# Autodesk Inventor assembly: 217-2792-001 Rev1
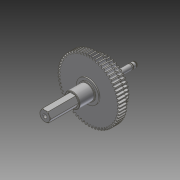
[picture p0: Inventor's stored thumbnail of the model, 180x180]
Saved by Autodesk Inventor 2014 SP1 (Build 180222100, 222)
## iProperties
Created: 2014-01-07
Part Number: 217-2792-001 Rev1
Document SubType Name: Assembly
Designer: Andrew Toennies
Mass: 632.627 g
Surface Area: 385.478 cm^2
Volume: 81.2914 cm^3
Density: 7.78222 g/cm^3
Author: Andrew Toennies
## Documents named in this file (7)
- C:\Users\Moses\Documents\GitHub\2014buildCAD\Shooter\Constrained 2 Speed Ball Shifter\217-2792-001 Rev1.iam
- C:\Users\Moses\Documents\GitHub\2014buildCAD\Shooter\Constrained 2 Speed Ball Shifter\217-2428-008 Rev1.ipt
- C:\Users\Moses\Documents\GitHub\2014buildCAD\Shooter\Constrained 2 Speed Ball Shifter\217-2428-028 Rev1_97633A250.ipt
- C:\Users\Moses\Documents\GitHub\2014buildCAD\Shooter\Constrained 2 Speed Ball Shifter\217-2709-101 Rev1.iam
- C:\Users\Moses\Documents\GitHub\2014buildCAD\Shooter\Constrained 2 Speed Ball Shifter\217-2713-101 Rev1.iam
- C:\Users\Moses\Documents\GitHub\2014buildCAD\Shooter\Constrained 2 Speed Ball Shifter\217-2790-001 Rev2.iam
- C:\Users\Moses\Documents\GitHub\2014buildCAD\Shooter\Constrained 2 Speed Ball Shifter\217-2428-007 Rev1.ipt
## Components (11 placed, 11 different names)
1. 217-2428-008 Rev1_55 — Insert:1, Insert:2
2. 217-2428-028 Rev1_97633A250_56 — Mate:1, Mate:2
3. 217-2709-101 Rev1_57 [sub-assembly] — Insert:1, Insert:3, High Speed Rotation
4. 217-2713-101 Rev1_58 [sub-assembly] — Insert:3, Mate:1, Low Speed Rotation
5. 217-2790-001 Rev2_59 [sub-assembly] — Insert:2, Mate:2, Low Speed Rotation, High Speed Rotation
6. 217-2428-007 Rev1_60
7. 217-2428-007 Rev1_61
8. 217-2428-007 Rev1_62
9. 217-2428-007 Rev1_63
10. 217-2428-007 Rev1_64
11. 217-2428-007 Rev1_65
## Relationships (7: Insert 3, Mate 2, RelateRotation 2)
- Insert:1: 217-2428-008 Rev1_55 ↔ 217-2709-101 Rev1_57
- Insert:2: 217-2428-008 Rev1_55 ↔ 217-2790-001 Rev2_59
- Insert:3: 217-2709-101 Rev1_57 ↔ 217-2713-101 Rev1_58
- Mate:1 (0.127 mm): 217-2428-028 Rev1_97633A250_56 ↔ 217-2713-101 Rev1_58
- Mate:2: 217-2428-028 Rev1_97633A250_56 ↔ 217-2790-001 Rev2_59
- Low Speed Rotation [RelateRotation] (1 ul): 217-2713-101 Rev1_58 ↔ 217-2790-001 Rev2_59
- High Speed Rotation [RelateRotation] (1 ul): 217-2709-101 Rev1_57 ↔ 217-2790-001 Rev2_59
